# Autodesk Inventor assembly: Room
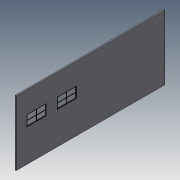
[picture p0: Inventor's stored thumbnail of the model, 180x180]
Saved by Autodesk Inventor 2018.3 (Build 223284000, 284)
## iProperties
Created: 2019-11-07
Part Number: Room
Document SubType Name: Assembly
Designer: MattBussey
Author: MattBussey
## Documents named in this file (3)
- C:\AVAInvAPI\Workspace\Assets\Room.iam
- C:\AVAInvAPI\Workspace\Assets\Wall.ipt
- C:\AVAInvAPI\Workspace\Assets\Window.ipt
## Components (3 placed, 2 different names)
1. Wall:1 — Mate:1, Mate:2, Flush:1, Mate:3, Mate:4, Flush:2
2. Window:1 — Mate:1, Mate:2, Flush:1
3. Window:2 — Mate:3, Mate:4, Flush:2
## Relationships (6: Mate 4, Flush 2)
- Mate:1: Wall:1 ↔ Window:1
- Mate:2: Wall:1 ↔ Window:1
- Flush:1: Wall:1 ↔ Window:1
- Mate:3: Wall:1 ↔ Window:2
- Mate:4: Wall:1 ↔ Window:2
- Flush:2: Wall:1 ↔ Window:2
